# Autodesk Inventor assembly: Full_assembly
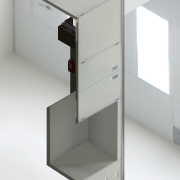
[picture p0: Inventor's stored thumbnail of the model, 180x180]
Saved by Autodesk Inventor 2016 SP2 (Build 200236200, 236)
## iProperties
Created: 2017-09-10
Part Number: Full_assembly
Document SubType Name: Assembly
Designer: Admin
Mass: 16830.8 g
Surface Area: 37966.6 cm^2
Volume: 18337.1 cm^3
Density: 0.917853 g/cm^3
Author: Admin
## Documents named in this file (4)
- E:\DATA\Inventor\AtongJali_v2\Full_assembly.iam
- E:\DATA\Inventor\AtongJali_v2\Gantry_y.iam
- E:\DATA\Inventor\AtongJali_v2\gantry_x.iam
- E:\DATA\Inventor\AtongJali_v2\NEMA23.ipt
## Components (3 placed, 3 different names)
1. Gantry_y:1 [sub-assembly] — Rigid:1
2. gantry_x:1 [sub-assembly] — Rigid:1
3. NEMA23:1
## Relationships (1: WeldJoint 1)
- Rigid:1 [WeldJoint]: Gantry_y:1 ↔ gantry_x:1
